# Autodesk Inventor assembly: worm_gear
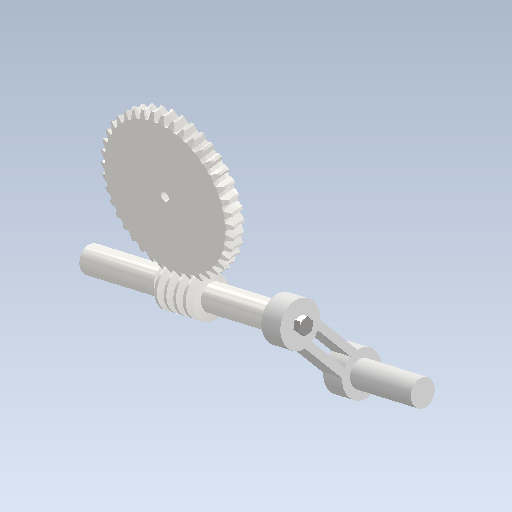
[picture p0: Inventor's stored thumbnail of the model, 512x512]
Saved by Autodesk Inventor 2020 (Build 240168000, 168)
## iProperties
Created: 2020-05-17
Part Number: worm_gear
Document SubType Name: Assembly
Designer: Hesekiel
Author: Hesekiel
## Documents named in this file (5)
- C:\Users\Hesekiel\Desktop\Equatorial-Mount-MUM\Mechanika\Mechanizm elewacji Filip\CAD\worm_gear.iam
- C:\Users\Hesekiel\Desktop\Equatorial-Mount-MUM\Mechanika\Mechanizm elewacji Filip\CAD\worm_gear\Design Accelerator\Worm Gears1.iam
- C:\Users\Hesekiel\Desktop\Equatorial-Mount-MUM\Mechanika\Mechanizm elewacji Filip\CAD\ramię_korby.ipt
- C:\Users\Hesekiel\Desktop\Equatorial-Mount-MUM\Mechanika\Mechanizm elewacji Filip\CAD\rączka_korby.ipt
- C:\Users\Hesekiel\Desktop\Equatorial-Mount-MUM\Mechanika\Mechanizm elewacji Filip\CAD\M10x30.ipt
## Components (5 placed, 4 different names)
1. Worm Gears:1 [sub-assembly] — Rigid:3
2. ramię_korby:1 — Rigid:2, Rigid:3, Rigid:4, Rigid:5
3. rączka_korby:1 — Rigid:2
4. M10x30:1 — Rigid:5
5. M10x30:2 — Rigid:4
## Relationships (4: WeldJoint 4)
- Rigid:2 [WeldJoint]: ramię_korby:1 ↔ rączka_korby:1
- Rigid:3 [WeldJoint]: Worm Gears:1 ↔ ramię_korby:1
- Rigid:4 [WeldJoint]: ramię_korby:1 ↔ M10x30:2
- Rigid:5 [WeldJoint]: ramię_korby:1 ↔ M10x30:1
